# Autodesk Inventor assembly: Ensemble1
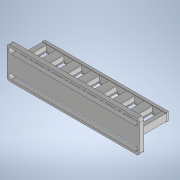
[picture p0: Inventor's stored thumbnail of the model, 180x180]
Saved by Autodesk Inventor 2020 (Build 240168000, 168)
## iProperties
Created: 2023-04-05
Part Number: Ensemble1
Document SubType Name: Assembly
Designer: Admin
Author: Admin
## Documents named in this file (4)
- E:\projet mutil 2022\3D detail INVENTOR\Ensemble1.iam
- E:\projet mutil 2022\3D detail INVENTOR\supportDB15.ipt
- E:\projet mutil 2022\3D detail INVENTOR\rend.ipt
- E:\projet mutil 2022\3D detail INVENTOR\Pièce11.ipt
## Components (8 placed, 3 different names)
1. supportDB15:1 — Logement:1, Logement:2, Logement:3, Logement:4, Logement:5, Logement:6, Affleurement:1
2. rend:1 — Logement:2
3. rend:2 — Logement:3
4. rend:3 — Logement:5
5. rend:4 — Logement:4
6. rend:5 — Logement:6
7. rend:6 — Logement:1
8. Pièce11:1 — Affleurement:1
## Relationships (7: Insert 6, Flush 1)
- Logement:1 [Insert]: supportDB15:1 ↔ rend:6
- Logement:2 [Insert]: supportDB15:1 ↔ rend:1
- Logement:3 [Insert]: supportDB15:1 ↔ rend:2
- Logement:4 [Insert]: supportDB15:1 ↔ rend:4
- Logement:5 [Insert]: supportDB15:1 ↔ rend:3
- Logement:6 [Insert]: supportDB15:1 ↔ rend:5
- Affleurement:1 [Flush]: supportDB15:1 ↔ Pièce11:1
